# Autodesk Inventor assembly: back support bearing and stopper.ipt
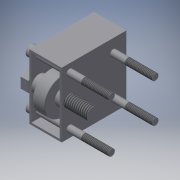
[picture p0: Inventor's stored thumbnail of the model, 180x180]
Saved by Autodesk Inventor 2018 (Build 220112000, 112)
## iProperties
Created: 2019-03-22
Part Number: back support bearing and stopper.ipt
Document SubType Name: Assembly
Designer: s-4008082
Author: s-4008082
## Documents named in this file (7)
- \\studenthome\students\S-4008082\robotics\back support bearing and stopper.ipt.iam
- \\studenthome\students\S-4008082\robotics\back support bearing holder.ipt
- \\studenthome\students\S-4008082\robotics\3 l 8 Bolt.ipt
- \\studenthome\students\S-4008082\robotics\10 l 20 2 1 l 2 bolt.ipt
- \\studenthome\students\S-4008082\robotics\1614zz bearing.ipt
- \\studenthome\students\S-4008082\robotics\.345 spacer.ipt
- \\studenthome\students\S-4008082\robotics\.15 spacer.ipt
## Components (9 placed, 6 different names)
1. back support bearing holder:1 — Mate:1, Mate:2, Mate:3, Mate:4, Mate:5, Mate:6, Mate:7, Mate:8, Mate:9, Mate:10, Mate:12, Mate:14, Mate:16
2. 3 l 8 Bolt:1 — Mate:9, Mate:10, Mate:11, Mate:13, Mate:15
3. 10 l 20 2 1 l 2 bolt:1 — Mate:5, Mate:6
4. 10 l 20 2 1 l 2 bolt:2 — Mate:3, Mate:4
5. 10 l 20 2 1 l 2 bolt:3 — Mate:7, Mate:8
6. 10 l 20 2 1 l 2 bolt:4 — Mate:1, Mate:2
7. 1614zz bearing:1 — Mate:11, Mate:12
8. .345 spacer:1 — Mate:15, Mate:16
9. .15 spacer:1 — Mate:13, Mate:14
## Relationships (16: Mate 16)
- Mate:1: back support bearing holder:1 ↔ 10 l 20 2 1 l 2 bolt:4
- Mate:2: back support bearing holder:1 ↔ 10 l 20 2 1 l 2 bolt:4
- Mate:3: back support bearing holder:1 ↔ 10 l 20 2 1 l 2 bolt:2
- Mate:4: back support bearing holder:1 ↔ 10 l 20 2 1 l 2 bolt:2
- Mate:5: back support bearing holder:1 ↔ 10 l 20 2 1 l 2 bolt:1
- Mate:6: back support bearing holder:1 ↔ 10 l 20 2 1 l 2 bolt:1
- Mate:7: back support bearing holder:1 ↔ 10 l 20 2 1 l 2 bolt:3
- Mate:8: back support bearing holder:1 ↔ 10 l 20 2 1 l 2 bolt:3
- Mate:9: back support bearing holder:1 ↔ 3 l 8 Bolt:1
- Mate:10: back support bearing holder:1 ↔ 3 l 8 Bolt:1
- Mate:11: 3 l 8 Bolt:1 ↔ 1614zz bearing:1
- Mate:12 (3.81 mm): back support bearing holder:1 ↔ 1614zz bearing:1
- Mate:13: 3 l 8 Bolt:1 ↔ .15 spacer:1
- Mate:14: back support bearing holder:1 ↔ .15 spacer:1
- Mate:15: 3 l 8 Bolt:1 ↔ .345 spacer:1
- Mate:16: back support bearing holder:1 ↔ .345 spacer:1
